# Autodesk Inventor assembly: Racks
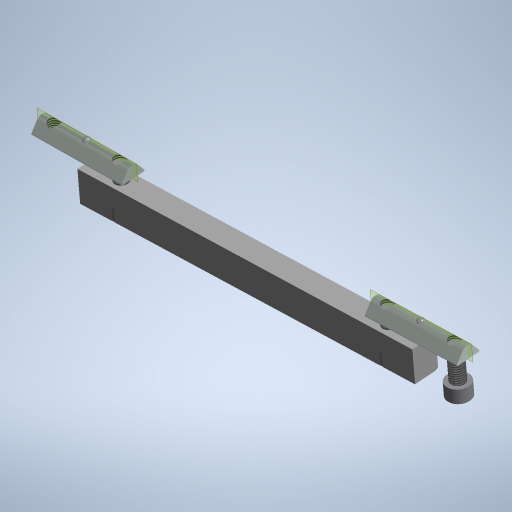
[picture p0: Inventor's stored thumbnail of the model, 512x512]
Saved by Autodesk Inventor 2023 (Build 270158000, 158)
## iProperties
Created: 2022-01-27
Part Number: Racks
Document SubType Name: Assembly
Designer: Elia
Author: Elia
## Documents named in this file (4)
- C:\Users\utente\OneDrive\Documenti\UniTN\I semestre\Mechanical Design\MDM-CyberOrto-CAD\Racks.iam
- C:\Users\utente\OneDrive\Documenti\UniTN\I semestre\Mechanical Design\MDM-CyberOrto-CAD\Rack_Pinion\Rack gear scaled1.ipt
- C:\Users\utente\OneDrive\Documenti\UniTN\I semestre\Mechanical Design\MDM-CyberOrto-CAD\Parker components\02-Fasteners\10-Standard T-Nuts\20-050.ipt
- C:\Users\utente\OneDrive\Documenti\UniTN\I semestre\Mechanical Design\MDM-CyberOrto-CAD\Parker components\02-Fasteners\16-Screws\01-Metric Screws\03-Socket Head\24-320-8SS.ipt
## Components (6 placed, 3 different names)
1. Rack gear scaled1:1 — Coincidente:2, Angolo:1, Allineato:4, Coincidente:6, Allineato:5, Allineato:6, Coincidente:8, Coincidente:9, Coincidente:14, Coincidente:15
2. 20-050:1 — Angolo:2, Allineato:3, Coincidente:5, Coincidente:6, Allineato:6
3. 20-050:2 — Allineato:5, Coincidente:16
4. 24-320-8SS:1 — Coincidente:8, Coincidente:9, Coincidente:16
5. 24-320-8SS:2 — Coincidente:14, Coincidente:15
6. 24-320-8SS:3
## Relationships (15: Mate 9, Flush 4, Angle 2)
- Coincidente:2 [Mate]: Rack gear scaled1:1
- Angolo:1 [Angle] (90 deg): Rack gear scaled1:1
- Angolo:2 [Angle] (90 deg): 20-050:1
- Allineato:3 [Flush] (-27.5 mm): 20-050:1
- Coincidente:4 [Mate]
- Allineato:4 [Flush] (-6.4645 mm): Rack gear scaled1:1
- Coincidente:5 [Mate]: 20-050:1
- Coincidente:6 [Mate]: Rack gear scaled1:1 ↔ 20-050:1
- Allineato:5 [Flush] (23.224 mm): Rack gear scaled1:1 ↔ 20-050:2
- Allineato:6 [Flush] (23.224 mm): Rack gear scaled1:1 ↔ 20-050:1
- Coincidente:8 [Mate]: Rack gear scaled1:1 ↔ 24-320-8SS:1
- Coincidente:9 [Mate]: Rack gear scaled1:1 ↔ 24-320-8SS:1
- Coincidente:14 [Mate]: Rack gear scaled1:1 ↔ 24-320-8SS:2
- Coincidente:15 [Mate]: Rack gear scaled1:1 ↔ 24-320-8SS:2
- Coincidente:16 [Mate]: 20-050:2 ↔ 24-320-8SS:1
